# Autodesk Inventor assembly: Lift.03.01.00.00
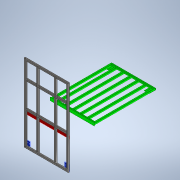
[picture p0: Inventor's stored thumbnail of the model, 180x180]
Saved by Autodesk Inventor 2021 (Build 250183000, 183)
## iProperties
_SolveAssemblyDoc: Frame Generator Solve Assembly
_Version: 25.0.0
Created: 2020-09-20
Part Number: Lift.03.01.00.00
Document SubType Name: Assembly
Designer: Kostya
Author: Kostya
## Documents named in this file (6)
- C:\Lift\Lift.03.01.00.00.iam
- C:\Lift\Lift.03.01.02.00.ipt
- C:\Lift\Lift.03.01.00.00\Frame\Frame 1600622124454.iam
- C:\Lift\Lift.03.01.01.00.iam
- C:\Lift\Lift.03.01.00.03.ipt
- C:\Lift\Lift.03.01.00.02_MIR.ipt
## Components (6 placed, 5 different names)
1. Lift.03.01.02.00:1
2. Frame 1600622124454:1 [sub-assembly] — Заподлицо:1, Совмещение:1, Заподлицо:3, Заподлицо:4, Заподлицо:5, Совмещение:2, Заподлицо:6, Совмещение:3, Заподлицо:7, Заподлицо:8
3. Lift.03.01.01.00:1 [sub-assembly] — Заподлицо:1
4. Lift.03.01.00.03:1 — Совмещение:1, Заподлицо:3
5. Lift.03.01.00.02_MIR:1 — Заподлицо:4, Заподлицо:5, Совмещение:2
6. Lift.03.01.00.02_MIR:2 — Совмещение:3, Заподлицо:7, Заподлицо:8
## Relationships (10: Flush 7, Mate 3)
- Заподлицо:1 [Flush]: Frame 1600622124454:1 ↔ Lift.03.01.01.00:1
- Совмещение:1 [Mate]: Frame 1600622124454:1 ↔ Lift.03.01.00.03:1
- Заподлицо:3 [Flush]: Frame 1600622124454:1 ↔ Lift.03.01.00.03:1
- Заподлицо:4 [Flush]: Frame 1600622124454:1 ↔ Lift.03.01.00.02_MIR:1
- Заподлицо:5 [Flush]: Frame 1600622124454:1 ↔ Lift.03.01.00.02_MIR:1
- Совмещение:2 [Mate]: Frame 1600622124454:1 ↔ Lift.03.01.00.02_MIR:1
- Заподлицо:6 [Flush] (-920 mm): Frame 1600622124454:1
- Совмещение:3 [Mate]: Frame 1600622124454:1 ↔ Lift.03.01.00.02_MIR:2
- Заподлицо:7 [Flush]: Frame 1600622124454:1 ↔ Lift.03.01.00.02_MIR:2
- Заподлицо:8 [Flush]: Frame 1600622124454:1 ↔ Lift.03.01.00.02_MIR:2
